# Autodesk Inventor assembly: DribblerUnit
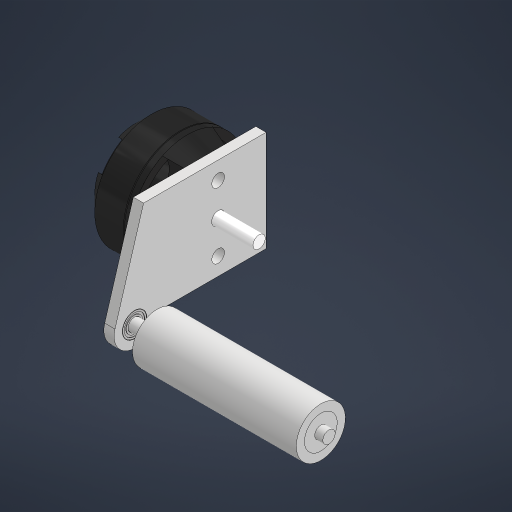
[picture p0: Inventor's stored thumbnail of the model, 512x512]
Saved by Autodesk Inventor 2024.2 (Build 282272000, 272)
## iProperties
Created: 2023-12-27
Part Number: DribblerUnit
Document SubType Name: Assembly
Designer: Hanaoka
Author: Hanaoka
## Documents named in this file (7)
- G:\共有ドライブ\reRo\05_個人\hanaoka\inventor\DribblerUnit\DribblerUnit.iam
- G:\共有ドライブ\reRo\05_個人\hanaoka\inventor\DribblerUnit\Dribbler_Tube.ipt
- G:\共有ドライブ\reRo\05_個人\hanaoka\inventor\DribblerUnit\C2822_BLDC\C2822_BLDC.ipt
- G:\共有ドライブ\reRo\05_個人\hanaoka\inventor\DribblerUnit\Gear_Frame.ipt
- G:\共有ドライブ\reRo\05_個人\hanaoka\inventor\DribblerUnit\Shaft_350.ipt
- G:\共有ドライブ\reRo\05_個人\hanaoka\inventor\DribblerUnit\Bearing_C-FL673ZZ\Bearing_C-FL673ZZ.ipt
- G:\共有ドライブ\reRo\05_個人\hanaoka\inventor\DribblerUnit\Tube_Hub.ipt
## Components (6 placed, 6 different names)
1. Dribbler_Tube:1 — 挿入:2
2. C2822_BLDC:1 — メイト:1, メイト:2, メイト:3
3. Gear_Frame:1 — 挿入:3, メイト:1, メイト:2, メイト:3, メイト:4, 正接:1, メイト:5
4. Shaft_350:1 — 挿入:1, 挿入:4
5. Bearing_C-FL673ZZ:1 — 挿入:1, 挿入:3
6. Tube_Hub:1 — 挿入:2, 挿入:4
## Relationships (10: Mate 5, Insert 4, Tangent 1)
- 挿入:1 [Insert]: Shaft_350:1 ↔ Bearing_C-FL673ZZ:1
- 挿入:2 [Insert]: Dribbler_Tube:1 ↔ Tube_Hub:1
- 挿入:3 [Insert]: Gear_Frame:1 ↔ Bearing_C-FL673ZZ:1
- 挿入:4 [Insert] (8 mm): Shaft_350:1 ↔ Tube_Hub:1
- メイト:1 [Mate]: C2822_BLDC:1 ↔ Gear_Frame:1
- メイト:2 [Mate]: C2822_BLDC:1 ↔ Gear_Frame:1
- メイト:3 [Mate]: C2822_BLDC:1 ↔ Gear_Frame:1
- メイト:4 [Mate]: Gear_Frame:1
- 正接:1 [Tangent]: Gear_Frame:1
- メイト:5 [Mate]: Gear_Frame:1
